# Autodesk Inventor assembly: КВ33.044.000
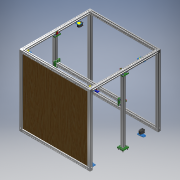
[picture p0: Inventor's stored thumbnail of the model, 180x180]
Saved by Autodesk Inventor 2019 (Build 230136000, 136)
## iProperties
Created: 2019-07-15
Part Number: КВ33.044.000
Material: Типовые
Document SubType Name: Assembly
Designer: Петров Иван
Description: Сортирующая ячейка
Author: Петров Иван
## Documents named in this file (13)
- E:\IVAN\Kvantoriada2019\optimal_gripper\hardware\КВ33.044.000 - Сортирующая ячейка.iam
- E:\IVAN\Kvantoriada2019\optimal_gripper\hardware\Стандартные изделия\Профиль станочный 30x30x740.ipt
- E:\IVAN\Kvantoriada2019\optimal_gripper\hardware\Стандартные изделия\Угол соединительный 30х30х30.ipt
- E:\IVAN\Kvantoriada2019\optimal_gripper\hardware\КВ33.044.001 - Дно.ipt
- E:\IVAN\Kvantoriada2019\optimal_gripper\hardware\КВ33.044.400 - Сборка деражтеля катка 6 мм.iam
- E:\IVAN\Kvantoriada2019\optimal_gripper\hardware\КВ33.044.200 - Каретка оси Х.iam
- E:\IVAN\Kvantoriada2019\optimal_gripper\hardware\Стандартные изделия\Профиль станочный 30x30x717.ipt
- E:\IVAN\Kvantoriada2019\optimal_gripper\hardware\КВ33.044.500 - Каретка оси Y.iam
- E:\IVAN\Kvantoriada2019\optimal_gripper\hardware\КВ33.044.301 - Деражатель мотора.ipt
- E:\IVAN\Kvantoriada2019\optimal_gripper\hardware\Стандартные изделия\Сервомотор Dynamixel AX-12A\ax-12a.iam
- E:\IVAN\Kvantoriada2019\optimal_gripper\hardware\колесо.ipt
- E:\IVAN\Kvantoriada2019\optimal_gripper\hardware\шкив.ipt
- E:\IVAN\Kvantoriada2019\optimal_gripper\hardware\проставка.ipt
## Components (46 placed, 12 different names)
1. КВ33.044.001 - Дно:1 — Совмещение:65, Совмещение:66, Совмещение:67
2. Профиль станочный 30x30x740:1 — Заподлицо:9, Заподлицо:10, Совмещение:4, Заподлицо:12, Совмещение:9, Заподлицо:17
3. Профиль станочный 30x30x740:2 — Совмещение:3, Заподлицо:2, Заподлицо:3, Совмещение:66, Совмещение:67, Совмещение:105
4. Профиль станочный 30x30x740:3 — Совмещение:1, Заподлицо:1, Заподлицо:5, Заподлицо:6, Заподлицо:8, Совмещение:5, Совмещение:65, Совмещение:109
5. Профиль станочный 30x30x740:4 — Заподлицо:14, Совмещение:7, Заподлицо:16, Заподлицо:18, Заподлицо:19, Совмещение:10, Совмещение:100, Совмещение:113
6. Угол соединительный 30х30х30:1 — Совмещение:1, Совмещение:2, Совмещение:3, Заподлицо:1, Заподлицо:2, Заподлицо:3, Заподлицо:4, Заподлицо:5, Заподлицо:38
7. Угол соединительный 30х30х30:2 — Заподлицо:18, Заподлицо:19, Совмещение:10, Совмещение:11, Заподлицо:20, Заподлицо:21
8. Угол соединительный 30х30х30:3 — Заподлицо:6, Заподлицо:7, Заподлицо:8, Заподлицо:9, Заподлицо:10, Совмещение:4, Заподлицо:11, Совмещение:5, Совмещение:6
9. Угол соединительный 30х30х30:4 — Заподлицо:12, Заподлицо:13, Заподлицо:14, Заподлицо:15, Совмещение:7, Совмещение:8, Заподлицо:16, Совмещение:9, Заподлицо:17
10. Профиль станочный 30x30x740:9 — Заподлицо:7, Заподлицо:11, Совмещение:6, Совмещение:19, Заподлицо:36, Заподлицо:37, Совмещение:108, Заподлицо:46, Совмещение:116, Совмещение:117, Совмещение:134, Заподлицо:55
11. Профиль станочный 30x30x740:10 — Заподлицо:13, Заподлицо:15, Совмещение:8, Совмещение:112, Заподлицо:48, Совмещение:114, Совмещение:115, Заподлицо:56, Совмещение:137
12. Профиль станочный 30x30x740:11 — Совмещение:11, Заподлицо:20, Заподлицо:21, Совмещение:101, Заподлицо:42, Совмещение:120, Совмещение:121, Совмещение:138, Заподлицо:58
13. Профиль станочный 30x30x740:12 — Совмещение:2, Заподлицо:4, Заподлицо:38, Совмещение:104, Заподлицо:44, Совмещение:118, Совмещение:119, Совмещение:140, Заподлицо:57
14. Профиль станочный 30x30x740:15 — Совмещение:135, Совмещение:136
15. Профиль станочный 30x30x740:16 — Совмещение:139, Совмещение:141
16. Профиль станочный 30x30x740:17
17. Профиль станочный 30x30x740:18
18. Угол соединительный 30х30х30:5
19. Угол соединительный 30х30х30:6
20. Угол соединительный 30х30х30:7 — Совмещение:19, Заподлицо:36, Заподлицо:37
21. Угол соединительный 30х30х30:8
22. КВ33.044.400 - Сборка деражтеля катка 6 мм:6 [sub-assembly] — Совмещение:100, Совмещение:101, Заподлицо:42
23. КВ33.044.400 - Сборка деражтеля катка 6 мм:7 [sub-assembly] — Совмещение:104, Заподлицо:44, Совмещение:105
24. КВ33.044.400 - Сборка деражтеля катка 6 мм:9 [sub-assembly] — Совмещение:108, Совмещение:109, Заподлицо:46
25. КВ33.044.400 - Сборка деражтеля катка 6 мм:10 [sub-assembly] — Совмещение:112, Заподлицо:48, Совмещение:113
26. КВ33.044.200 - Каретка оси Х:1 [sub-assembly] — Совмещение:114, Совмещение:115, Совмещение:122, Заподлицо:49, Заподлицо:50
27. КВ33.044.200 - Каретка оси Х:2 [sub-assembly] — Совмещение:116, Совмещение:117, Совмещение:123
28. КВ33.044.200 - Каретка оси Х:3 [sub-assembly] — Совмещение:118, Совмещение:119, Совмещение:124, Совмещение:125
29. КВ33.044.200 - Каретка оси Х:4 [sub-assembly] — Совмещение:120, Совмещение:121, Заподлицо:51, Заподлицо:52
30. КВ33.044.200 - Каретка оси Х:5 [sub-assembly] — Совмещение:126, Совмещение:127, Совмещение:131
31. КВ33.044.200 - Каретка оси Х:6 [sub-assembly] — Совмещение:128, Совмещение:129, Заподлицо:53, Совмещение:130, Заподлицо:54
32. КВ33.044.500 - Каретка оси Y:1 [sub-assembly] — Совмещение:132, Совмещение:133
33. Профиль станочный 30x30x717:3 — Заподлицо:53, Совмещение:130, Заподлицо:54, Совмещение:131, Совмещение:132, Совмещение:133
34. Профиль станочный 30x30x717:1 — Совмещение:122, Заподлицо:49, Заподлицо:50, Совмещение:123, Совмещение:126, Совмещение:127
35. Профиль станочный 30x30x717:2 — Заподлицо:51, Заподлицо:52, Совмещение:124, Совмещение:125, Совмещение:128, Совмещение:129
36. КВ33.044.301 - Деражатель мотора:1 — Совмещение:134, Совмещение:135, Заподлицо:55, Совмещение:151, Совмещение:152, Совмещение:153
37. КВ33.044.301 - Деражатель мотора:2 — Совмещение:140, Совмещение:141, Заподлицо:57, Совмещение:148, Совмещение:149, Совмещение:150
38. КВ33.044.301 - Деражатель мотора:3 — Совмещение:138, Совмещение:139, Совмещение:145, Заподлицо:58, Совмещение:146, Совмещение:147
39. КВ33.044.301 - Деражатель мотора:4 — Совмещение:136, Заподлицо:56, Совмещение:137, Совмещение:142, Совмещение:143, Совмещение:144
40. ax-12a:1 [sub-assembly] — Совмещение:142, Совмещение:143, Совмещение:144
41. ax-12a:2 [sub-assembly] — Совмещение:151, Совмещение:152, Совмещение:153
42. ax-12a:3 [sub-assembly] — Совмещение:148, Совмещение:149, Совмещение:150
43. ax-12a:4 [sub-assembly] — Совмещение:145, Совмещение:146, Совмещение:147, Совмещение:154, Совмещение:155, Совмещение:159, Совмещение:160
44. колесо:1 — Совмещение:154, Совмещение:155, Совмещение:156, Совмещение:157, Совмещение:158
45. шкив:1 — Совмещение:156, Совмещение:157, Совмещение:158
46. проставка:1 — Совмещение:159, Совмещение:160
## Relationships (129: Mate 77, Flush 52)
- Совмещение:1 [Mate]: Профиль станочный 30x30x740:3 ↔ Угол соединительный 30х30х30:1
- Совмещение:2 [Mate]: Угол соединительный 30х30х30:1 ↔ Профиль станочный 30x30x740:12
- Совмещение:3 [Mate]: Профиль станочный 30x30x740:2 ↔ Угол соединительный 30х30х30:1
- Заподлицо:1 [Flush]: Профиль станочный 30x30x740:3 ↔ Угол соединительный 30х30х30:1
- Заподлицо:2 [Flush]: Профиль станочный 30x30x740:2 ↔ Угол соединительный 30х30х30:1
- Заподлицо:3 [Flush]: Профиль станочный 30x30x740:2 ↔ Угол соединительный 30х30х30:1
- Заподлицо:4 [Flush]: Угол соединительный 30х30х30:1 ↔ Профиль станочный 30x30x740:12
- Заподлицо:5 [Flush]: Профиль станочный 30x30x740:3 ↔ Угол соединительный 30х30х30:1
- Заподлицо:6 [Flush]: Профиль станочный 30x30x740:3 ↔ Угол соединительный 30х30х30:3
- Заподлицо:7 [Flush]: Угол соединительный 30х30х30:3 ↔ Профиль станочный 30x30x740:9
- Заподлицо:8 [Flush]: Профиль станочный 30x30x740:3 ↔ Угол соединительный 30х30х30:3
- Заподлицо:9 [Flush]: Профиль станочный 30x30x740:1 ↔ Угол соединительный 30х30х30:3
- Заподлицо:10 [Flush]: Профиль станочный 30x30x740:1 ↔ Угол соединительный 30х30х30:3
- Совмещение:4 [Mate]: Профиль станочный 30x30x740:1 ↔ Угол соединительный 30х30х30:3
- Заподлицо:11 [Flush]: Угол соединительный 30х30х30:3 ↔ Профиль станочный 30x30x740:9
- Совмещение:5 [Mate]: Профиль станочный 30x30x740:3 ↔ Угол соединительный 30х30х30:3
- Совмещение:6 [Mate]: Угол соединительный 30х30х30:3 ↔ Профиль станочный 30x30x740:9
- Заподлицо:12 [Flush]: Профиль станочный 30x30x740:1 ↔ Угол соединительный 30х30х30:4
- Заподлицо:13 [Flush]: Угол соединительный 30х30х30:4 ↔ Профиль станочный 30x30x740:10
- Заподлицо:14 [Flush]: Профиль станочный 30x30x740:4 ↔ Угол соединительный 30х30х30:4
- Заподлицо:15 [Flush]: Угол соединительный 30х30х30:4 ↔ Профиль станочный 30x30x740:10
- Совмещение:7 [Mate]: Профиль станочный 30x30x740:4 ↔ Угол соединительный 30х30х30:4
- Совмещение:8 [Mate]: Угол соединительный 30х30х30:4 ↔ Профиль станочный 30x30x740:10
- Заподлицо:16 [Flush]: Профиль станочный 30x30x740:4 ↔ Угол соединительный 30х30х30:4
- Совмещение:9 [Mate]: Профиль станочный 30x30x740:1 ↔ Угол соединительный 30х30х30:4
- Заподлицо:17 [Flush]: Профиль станочный 30x30x740:1 ↔ Угол соединительный 30х30х30:4
- Заподлицо:18 [Flush]: Профиль станочный 30x30x740:4 ↔ Угол соединительный 30х30х30:2
- Заподлицо:19 [Flush]: Профиль станочный 30x30x740:4 ↔ Угол соединительный 30х30х30:2
- Совмещение:10 [Mate]: Профиль станочный 30x30x740:4 ↔ Угол соединительный 30х30х30:2
- Совмещение:11 [Mate]: Угол соединительный 30х30х30:2 ↔ Профиль станочный 30x30x740:11
- Заподлицо:20 [Flush]: Угол соединительный 30х30х30:2 ↔ Профиль станочный 30x30x740:11
- Заподлицо:21 [Flush]: Угол соединительный 30х30х30:2 ↔ Профиль станочный 30x30x740:11
- [Mate]: Профиль станочный 30x30x740:17 ↔ Угол соединительный 30х30х30:5
- [Mate]: Профиль станочный 30x30x740:16 ↔ Угол соединительный 30х30х30:5
- [Flush]: Профиль станочный 30x30x740:17 ↔ Угол соединительный 30х30х30:5
- [Flush]: Профиль станочный 30x30x740:16 ↔ Угол соединительный 30х30х30:5
- [Flush]: Профиль станочный 30x30x740:16 ↔ Угол соединительный 30х30х30:5
- [Flush]: Профиль станочный 30x30x740:17 ↔ Угол соединительный 30х30х30:5
- [Flush]: Профиль станочный 30x30x740:17 ↔ Угол соединительный 30х30х30:7
- [Flush]: Профиль станочный 30x30x740:17 ↔ Угол соединительный 30х30х30:7
- [Flush]: Профиль станочный 30x30x740:15 ↔ Угол соединительный 30х30х30:7
- [Flush]: Профиль станочный 30x30x740:15 ↔ Угол соединительный 30х30х30:7
- [Mate]: Профиль станочный 30x30x740:15 ↔ Угол соединительный 30х30х30:7
- [Mate]: Профиль станочный 30x30x740:17 ↔ Угол соединительный 30х30х30:7
- [Flush]: Профиль станочный 30x30x740:15 ↔ Угол соединительный 30х30х30:8
- [Flush]: Профиль станочный 30x30x740:18 ↔ Угол соединительный 30х30х30:8
- [Mate]: Профиль станочный 30x30x740:18 ↔ Угол соединительный 30х30х30:8
- [Flush]: Профиль станочный 30x30x740:18 ↔ Угол соединительный 30х30х30:8
- [Mate]: Профиль станочный 30x30x740:15 ↔ Угол соединительный 30х30х30:8
- [Flush]: Профиль станочный 30x30x740:15 ↔ Угол соединительный 30х30х30:8
- [Flush]: Профиль станочный 30x30x740:18 ↔ Угол соединительный 30х30х30:6
- [Flush]: Профиль станочный 30x30x740:18 ↔ Угол соединительный 30х30х30:6
- [Mate]: Профиль станочный 30x30x740:18 ↔ Угол соединительный 30х30х30:6
- Совмещение:19 [Mate]: Профиль станочный 30x30x740:9 ↔ Угол соединительный 30х30х30:7
- Заподлицо:36 [Flush]: Профиль станочный 30x30x740:9 ↔ Угол соединительный 30х30х30:7
- Заподлицо:37 [Flush]: Профиль станочный 30x30x740:9 ↔ Угол соединительный 30х30х30:7
- Заподлицо:38 [Flush]: Угол соединительный 30х30х30:1 ↔ Профиль станочный 30x30x740:12
- Совмещение:65 [Mate]: КВ33.044.001 - Дно:1 ↔ Профиль станочный 30x30x740:3
- Совмещение:66 [Mate]: КВ33.044.001 - Дно:1 ↔ Профиль станочный 30x30x740:2
- Совмещение:67 [Mate]: КВ33.044.001 - Дно:1 ↔ Профиль станочный 30x30x740:2
- Совмещение:100 [Mate]: Профиль станочный 30x30x740:4 ↔ КВ33.044.400 - Сборка деражтеля катка 6 мм:6
- Совмещение:101 [Mate]: Профиль станочный 30x30x740:11 ↔ КВ33.044.400 - Сборка деражтеля катка 6 мм:6
- Заподлицо:42 [Flush]: Профиль станочный 30x30x740:11 ↔ КВ33.044.400 - Сборка деражтеля катка 6 мм:6
- Совмещение:104 [Mate]: Профиль станочный 30x30x740:12 ↔ КВ33.044.400 - Сборка деражтеля катка 6 мм:7
- Заподлицо:44 [Flush]: Профиль станочный 30x30x740:12 ↔ КВ33.044.400 - Сборка деражтеля катка 6 мм:7
- Совмещение:105 [Mate]: Профиль станочный 30x30x740:2 ↔ КВ33.044.400 - Сборка деражтеля катка 6 мм:7
- Совмещение:108 [Mate]: Профиль станочный 30x30x740:9 ↔ КВ33.044.400 - Сборка деражтеля катка 6 мм:9
- Совмещение:109 [Mate]: Профиль станочный 30x30x740:3 ↔ КВ33.044.400 - Сборка деражтеля катка 6 мм:9
- Заподлицо:46 [Flush]: Профиль станочный 30x30x740:9 ↔ КВ33.044.400 - Сборка деражтеля катка 6 мм:9
- Совмещение:112 [Mate]: Профиль станочный 30x30x740:10 ↔ КВ33.044.400 - Сборка деражтеля катка 6 мм:10
- Заподлицо:48 [Flush]: Профиль станочный 30x30x740:10 ↔ КВ33.044.400 - Сборка деражтеля катка 6 мм:10
- Совмещение:113 [Mate]: Профиль станочный 30x30x740:4 ↔ КВ33.044.400 - Сборка деражтеля катка 6 мм:10
- Совмещение:114 [Mate] (1.5 mm): Профиль станочный 30x30x740:10 ↔ КВ33.044.200 - Каретка оси Х:1
- Совмещение:115 [Mate] (1.02 mm): Профиль станочный 30x30x740:10 ↔ КВ33.044.200 - Каретка оси Х:1
- Совмещение:116 [Mate] (1.5 mm): Профиль станочный 30x30x740:9 ↔ КВ33.044.200 - Каретка оси Х:2
- Совмещение:117 [Mate] (1.02 mm): Профиль станочный 30x30x740:9 ↔ КВ33.044.200 - Каретка оси Х:2
- Совмещение:118 [Mate] (1.5 mm): Профиль станочный 30x30x740:12 ↔ КВ33.044.200 - Каретка оси Х:3
- Совмещение:119 [Mate] (1.02 mm): Профиль станочный 30x30x740:12 ↔ КВ33.044.200 - Каретка оси Х:3
- Совмещение:120 [Mate] (1.5 mm): Профиль станочный 30x30x740:11 ↔ КВ33.044.200 - Каретка оси Х:4
- Совмещение:121 [Mate] (1.02 mm): Профиль станочный 30x30x740:11 ↔ КВ33.044.200 - Каретка оси Х:4
- Совмещение:122 [Mate]: КВ33.044.200 - Каретка оси Х:1 ↔ Профиль станочный 30x30x717:1
- Заподлицо:49 [Flush] (20 mm): КВ33.044.200 - Каретка оси Х:1 ↔ Профиль станочный 30x30x717:1
- Заподлицо:50 [Flush] (19 mm): КВ33.044.200 - Каретка оси Х:1 ↔ Профиль станочный 30x30x717:1
- Совмещение:123 [Mate]: КВ33.044.200 - Каретка оси Х:2 ↔ Профиль станочный 30x30x717:1
- Заподлицо:51 [Flush] (20 mm): КВ33.044.200 - Каретка оси Х:4 ↔ Профиль станочный 30x30x717:2
- Заподлицо:52 [Flush] (19 mm): КВ33.044.200 - Каретка оси Х:4 ↔ Профиль станочный 30x30x717:2
- Совмещение:124 [Mate]: КВ33.044.200 - Каретка оси Х:3 ↔ Профиль станочный 30x30x717:2
- Совмещение:125 [Mate]: КВ33.044.200 - Каретка оси Х:3 ↔ Профиль станочный 30x30x717:2
- Совмещение:126 [Mate] (1.02 mm): КВ33.044.200 - Каретка оси Х:5 ↔ Профиль станочный 30x30x717:1
- Совмещение:127 [Mate] (1.5 mm): КВ33.044.200 - Каретка оси Х:5 ↔ Профиль станочный 30x30x717:1
- Совмещение:128 [Mate] (1.02 mm): КВ33.044.200 - Каретка оси Х:6 ↔ Профиль станочный 30x30x717:2
- Совмещение:129 [Mate] (1.5 mm): КВ33.044.200 - Каретка оси Х:6 ↔ Профиль станочный 30x30x717:2
- Заподлицо:53 [Flush] (19 mm): КВ33.044.200 - Каретка оси Х:6 ↔ Профиль станочный 30x30x717:3
- Совмещение:130 [Mate]: КВ33.044.200 - Каретка оси Х:6 ↔ Профиль станочный 30x30x717:3
- Заподлицо:54 [Flush] (20 mm): КВ33.044.200 - Каретка оси Х:6 ↔ Профиль станочный 30x30x717:3
- Совмещение:131 [Mate]: КВ33.044.200 - Каретка оси Х:5 ↔ Профиль станочный 30x30x717:3
- Совмещение:132 [Mate] (1.5 mm): КВ33.044.500 - Каретка оси Y:1 ↔ Профиль станочный 30x30x717:3
- Совмещение:133 [Mate] (1.02 mm): КВ33.044.500 - Каретка оси Y:1 ↔ Профиль станочный 30x30x717:3
- Совмещение:134 [Mate]: Профиль станочный 30x30x740:9 ↔ КВ33.044.301 - Деражатель мотора:1
- Совмещение:135 [Mate] (130 mm): Профиль станочный 30x30x740:15 ↔ КВ33.044.301 - Деражатель мотора:1
- Заподлицо:55 [Flush]: Профиль станочный 30x30x740:9 ↔ КВ33.044.301 - Деражатель мотора:1
- Совмещение:136 [Mate] (130 mm): Профиль станочный 30x30x740:15 ↔ КВ33.044.301 - Деражатель мотора:4
- Заподлицо:56 [Flush]: Профиль станочный 30x30x740:10 ↔ КВ33.044.301 - Деражатель мотора:4
- Совмещение:137 [Mate]: Профиль станочный 30x30x740:10 ↔ КВ33.044.301 - Деражатель мотора:4
- Совмещение:138 [Mate]: Профиль станочный 30x30x740:11 ↔ КВ33.044.301 - Деражатель мотора:3
- Совмещение:139 [Mate] (130 mm): Профиль станочный 30x30x740:16 ↔ КВ33.044.301 - Деражатель мотора:3
- Совмещение:140 [Mate]: Профиль станочный 30x30x740:12 ↔ КВ33.044.301 - Деражатель мотора:2
- Совмещение:141 [Mate] (130 mm): Профиль станочный 30x30x740:16 ↔ КВ33.044.301 - Деражатель мотора:2
- Заподлицо:57 [Flush]: Профиль станочный 30x30x740:12 ↔ КВ33.044.301 - Деражатель мотора:2
- Совмещение:142 [Mate]: КВ33.044.301 - Деражатель мотора:4 ↔ ax-12a:1
- Совмещение:143 [Mate]: КВ33.044.301 - Деражатель мотора:4 ↔ ax-12a:1
- Совмещение:144 [Mate]: КВ33.044.301 - Деражатель мотора:4 ↔ ax-12a:1
- Совмещение:145 [Mate]: КВ33.044.301 - Деражатель мотора:3 ↔ ax-12a:4
- Заподлицо:58 [Flush]: Профиль станочный 30x30x740:11 ↔ КВ33.044.301 - Деражатель мотора:3
- Совмещение:146 [Mate]: КВ33.044.301 - Деражатель мотора:3 ↔ ax-12a:4
- Совмещение:147 [Mate]: КВ33.044.301 - Деражатель мотора:3 ↔ ax-12a:4
- Совмещение:148 [Mate]: КВ33.044.301 - Деражатель мотора:2 ↔ ax-12a:3
- Совмещение:149 [Mate]: КВ33.044.301 - Деражатель мотора:2 ↔ ax-12a:3
- Совмещение:150 [Mate]: КВ33.044.301 - Деражатель мотора:2 ↔ ax-12a:3
- Совмещение:151 [Mate]: КВ33.044.301 - Деражатель мотора:1 ↔ ax-12a:2
- Совмещение:152 [Mate]: КВ33.044.301 - Деражатель мотора:1 ↔ ax-12a:2
- Совмещение:153 [Mate]: КВ33.044.301 - Деражатель мотора:1 ↔ ax-12a:2
- Совмещение:154 [Mate]: ax-12a:4 ↔ колесо:1
- Совмещение:155 [Mate] (4 mm): ax-12a:4 ↔ колесо:1
- Совмещение:156 [Mate]: колесо:1 ↔ шкив:1
- Совмещение:157 [Mate]: колесо:1 ↔ шкив:1
- Совмещение:158 [Mate]: колесо:1 ↔ шкив:1
- Совмещение:159 [Mate]: ax-12a:4 ↔ проставка:1
- Совмещение:160 [Mate]: ax-12a:4 ↔ проставка:1
## Named parameters: d91_d80 = 0 mm, d92_d82 = 0 mm, d93_d83 = 0 mm, d94_d84 = 0 mm, d95_d85 = 0 mm, d96_d86 = 0 mm, d97_d87 = 0 mm, d98_d66 = 0 mm, d99_d67 = 0 mm, d100_d69 = 0 mm, d101_d70 = 0 mm, d102_d71 = 0 mm, d103_d72 = 0 mm, d104_d74 = 0 mm, d105_d76 = 0 mm, d106_d78 = 0 mm, d107_d59 = 0 mm, d108_d61 = 0 mm, d109_d62 = 0 mm, d110_d63 = 0 mm, d111_d64 = 0 mm
